# Autodesk Inventor assembly: PUERTA SP40-02 INT-EXT 2073x761
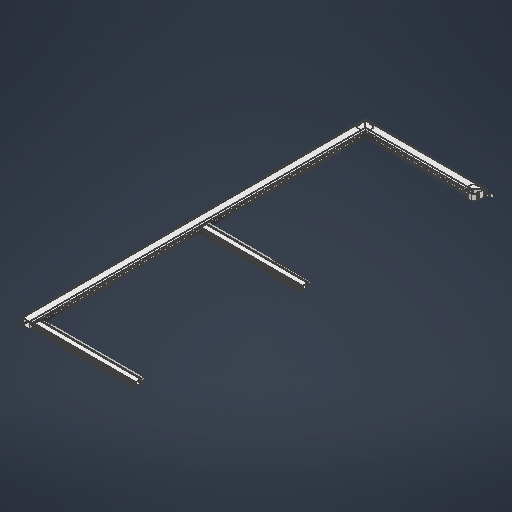
[picture p0: Inventor's stored thumbnail of the model, 512x512]
Saved by Autodesk Inventor 2025 (Build 290162000, 162)
## iProperties
Created: 2026-02-13
Part Number: PUERTA SP40-02 INT-EXT 2073x761
Document SubType Name: Assembly
Designer: ROLANDO
Author: ROLANDO
## Documents named in this file (16)
- C:\Users\rolan\OneDrive\Documentos\Inventor\Projects\CARPINTERIA ALUMINIO\PUERTAS Y VENTANAS\PUERTAS\PUERTA SP40-02 INT-EXT 2073x761.iam
- C:\Users\rolan\OneDrive\Documentos\Inventor\Projects\CARPINTERIA ALUMINIO\PUERTAS Y VENTANAS\PUERTAS\SP40-02 HOJA PUERTA BATIENTE INT - EXT 761 mm.ipt
- SP40-02 HOJA PUERTA BATIENTE INT - EXT 761 mm.ipt
- C:\Users\rolan\OneDrive\Documentos\Inventor\Projects\CARPINTERIA ALUMINIO\PUERTAS Y VENTANAS\PUERTAS\SP40-02 HOJA PUERTA BATIENTE INT - EXT 2073 mm.ipt
- SP40-02 HOJA PUERTA BATIENTE INT - EXT 2073 mm.ipt
- C:\Users\rolan\OneDrive\Documentos\Inventor\Projects\CARPINTERIA ALUMINIO\PUERTAS Y VENTANAS\ESCUADRAS\ESCUADRA UNIÓN 45 GRUESA.ipt
- C:\Users\rolan\OneDrive\Documentos\Inventor\Projects\CARPINTERIA ALUMINIO\PUERTAS Y VENTANAS\PUERTAS\SP40-02 JUNTA EXT 2073.ipt
- C:\Users\rolan\OneDrive\Documentos\Inventor\Projects\CARPINTERIA ALUMINIO\PUERTAS Y VENTANAS\PUERTAS\SP40-02 JUNTA EXT 761.ipt
- C:\Users\rolan\OneDrive\Documentos\Inventor\Projects\CARPINTERIA ALUMINIO\PUERTAS Y VENTANAS\PUERTAS\SP40-02 JUNTA INT 2073.ipt
- C:\Users\rolan\OneDrive\Documentos\Inventor\Projects\CARPINTERIA ALUMINIO\PUERTAS Y VENTANAS\PUERTAS\SP40-02 JUNTA INT 761.ipt
- C:\Users\rolan\OneDrive\Documentos\Inventor\Projects\CARPINTERIA ALUMINIO\PUERTAS Y VENTANAS\PUERTAS\SP40-02 HOJA PUERTA BATIENTE INT - EXT 2073 mm_MIR.ipt
- C:\Users\rolan\OneDrive\Documentos\Inventor\Projects\CARPINTERIA ALUMINIO\PUERTAS Y VENTANAS\PUERTAS\SP40-02 JUNTA EXT 2073_MIR.ipt
- C:\Users\rolan\OneDrive\Documentos\Inventor\Projects\CARPINTERIA ALUMINIO\PUERTAS Y VENTANAS\PUERTAS\SP40-02 JUNTA INT 2073_MIR.ipt
- C:\Users\rolan\OneDrive\Documentos\Inventor\Projects\CARPINTERIA ALUMINIO\PUERTAS Y VENTANAS\ESCUADRAS\ESCUADRA UNIÓN 45 GRUESA_MIR3.ipt
- C:\Users\rolan\OneDrive\Documentos\Inventor\Projects\CARPINTERIA ALUMINIO\PUERTAS Y VENTANAS\PUERTAS\SP40-04 TRAVESAÑO CENTRAL ZOCALO 602x60.ipt
- C:\Users\rolan\OneDrive\Documentos\Inventor\Projects\CARPINTERIA ALUMINIO\PUERTAS Y VENTANAS\PUERTAS\SP40-02 JUNTA INT 602 ZOCALO.ipt
## Components (16 placed, 13 different names)
1. SP40-02 HOJA PUERTA BATIENTE INT - EXT 761 mm:1 — Coincidencia:1, Coincidencia:3, Coincidencia:4, Coincidencia:5, Coincidencia:13, Coincidencia:14, Nivelación:5, Coincidencia:15, Coincidencia:16, Nivelación:6, Nivelación:9, Coincidencia:23, Coincidencia:25, Coincidencia:26, Coincidencia:29
2. SP40-02 HOJA PUERTA BATIENTE INT - EXT 2073 mm:1 — Coincidencia:2, Coincidencia:4, Coincidencia:5, Coincidencia:6, Coincidencia:7, Coincidencia:8, Nivelación:2, Coincidencia:11, Coincidencia:12, Nivelación:4
3. ESCUADRA UNIÓN 45 GRUESA:1 — Coincidencia:1, Coincidencia:2, Coincidencia:3, Coincidencia:6
4. SP40-02 JUNTA EXT 2073:1 — Coincidencia:7, Coincidencia:8, Nivelación:2
5. SP40-02 JUNTA EXT 761:1 — Coincidencia:15, Coincidencia:16, Nivelación:6
6. SP40-02 JUNTA INT 2073:1 — Coincidencia:11, Coincidencia:12, Nivelación:4
7. SP40-02 JUNTA INT 761:1 — Coincidencia:13, Coincidencia:14, Nivelación:5
8. SP40-02 HOJA PUERTA BATIENTE INT - EXT 2073 mm_MIR:1 — Coincidencia:18, Nivelación:7, Coincidencia:19, Coincidencia:20, Nivelación:8, Coincidencia:21, Coincidencia:22, Coincidencia:24, Coincidencia:25, Coincidencia:26, Coincidencia:27, Nivelación:10, Coincidencia:28, Nivelación:11, Nivelación:12
9. ESCUADRA UNIÓN 45 GRUESA_MIR3:1 — Nivelación:9, Coincidencia:18, Coincidencia:23, Coincidencia:24
10. SP40-02 JUNTA EXT 2073_MIR:1 — Nivelación:7, Coincidencia:19, Coincidencia:20
11. SP40-02 JUNTA INT 2073_MIR:1 — Nivelación:8, Coincidencia:21, Coincidencia:22
12. SP40-04 TRAVESAÑO CENTRAL ZOCALO 602x60:1 — Coincidencia:28, Nivelación:11, Nivelación:12, Coincidencia:30, Coincidencia:31, Nivelación:13
13. SP40-04 TRAVESAÑO CENTRAL ZOCALO 602x60:2 — Coincidencia:27, Nivelación:10, Coincidencia:29, Coincidencia:32, Coincidencia:33, Nivelación:14, Coincidencia:34, Coincidencia:35, Nivelación:15
14. SP40-02 JUNTA INT 602 ZOCALO:1 — Coincidencia:32, Coincidencia:33, Nivelación:14
15. SP40-02 JUNTA INT 602 ZOCALO:2 — Coincidencia:34, Coincidencia:35, Nivelación:15
16. SP40-02 JUNTA INT 602 ZOCALO:3 — Coincidencia:30, Coincidencia:31, Nivelación:13
## Relationships (45: Mate 32, Flush 13)
- Coincidencia:1 [Mate]: SP40-02 HOJA PUERTA BATIENTE INT - EXT 761 mm:1 ↔ ESCUADRA UNIÓN 45 GRUESA:1
- Coincidencia:2 [Mate]: SP40-02 HOJA PUERTA BATIENTE INT - EXT 2073 mm:1 ↔ ESCUADRA UNIÓN 45 GRUESA:1
- Coincidencia:3 [Mate] (0.2 mm): SP40-02 HOJA PUERTA BATIENTE INT - EXT 761 mm:1 ↔ ESCUADRA UNIÓN 45 GRUESA:1
- Coincidencia:4 [Mate]: SP40-02 HOJA PUERTA BATIENTE INT - EXT 761 mm:1 ↔ SP40-02 HOJA PUERTA BATIENTE INT - EXT 2073 mm:1
- Coincidencia:5 [Mate]: SP40-02 HOJA PUERTA BATIENTE INT - EXT 761 mm:1 ↔ SP40-02 HOJA PUERTA BATIENTE INT - EXT 2073 mm:1
- Coincidencia:6 [Mate] (0.1 mm): SP40-02 HOJA PUERTA BATIENTE INT - EXT 2073 mm:1 ↔ ESCUADRA UNIÓN 45 GRUESA:1
- Coincidencia:7 [Mate]: SP40-02 HOJA PUERTA BATIENTE INT - EXT 2073 mm:1 ↔ SP40-02 JUNTA EXT 2073:1
- Coincidencia:8 [Mate]: SP40-02 HOJA PUERTA BATIENTE INT - EXT 2073 mm:1 ↔ SP40-02 JUNTA EXT 2073:1
- Nivelación:2 [Flush]: SP40-02 HOJA PUERTA BATIENTE INT - EXT 2073 mm:1 ↔ SP40-02 JUNTA EXT 2073:1
- Coincidencia:11 [Mate]: SP40-02 HOJA PUERTA BATIENTE INT - EXT 2073 mm:1 ↔ SP40-02 JUNTA INT 2073:1
- Coincidencia:12 [Mate]: SP40-02 HOJA PUERTA BATIENTE INT - EXT 2073 mm:1 ↔ SP40-02 JUNTA INT 2073:1
- Nivelación:4 [Flush]: SP40-02 HOJA PUERTA BATIENTE INT - EXT 2073 mm:1 ↔ SP40-02 JUNTA INT 2073:1
- Coincidencia:13 [Mate]: SP40-02 HOJA PUERTA BATIENTE INT - EXT 761 mm:1 ↔ SP40-02 JUNTA INT 761:1
- Coincidencia:14 [Mate]: SP40-02 HOJA PUERTA BATIENTE INT - EXT 761 mm:1 ↔ SP40-02 JUNTA INT 761:1
- Nivelación:5 [Flush]: SP40-02 HOJA PUERTA BATIENTE INT - EXT 761 mm:1 ↔ SP40-02 JUNTA INT 761:1
- Coincidencia:15 [Mate]: SP40-02 HOJA PUERTA BATIENTE INT - EXT 761 mm:1 ↔ SP40-02 JUNTA EXT 761:1
- Coincidencia:16 [Mate]: SP40-02 HOJA PUERTA BATIENTE INT - EXT 761 mm:1 ↔ SP40-02 JUNTA EXT 761:1
- Nivelación:6 [Flush]: SP40-02 HOJA PUERTA BATIENTE INT - EXT 761 mm:1 ↔ SP40-02 JUNTA EXT 761:1
- Nivelación:9 [Flush]: SP40-02 HOJA PUERTA BATIENTE INT - EXT 761 mm:1 ↔ ESCUADRA UNIÓN 45 GRUESA_MIR3:1
- Coincidencia:18 [Mate]: SP40-02 HOJA PUERTA BATIENTE INT - EXT 2073 mm_MIR:1 ↔ ESCUADRA UNIÓN 45 GRUESA_MIR3:1
- Nivelación:7 [Flush]: SP40-02 HOJA PUERTA BATIENTE INT - EXT 2073 mm_MIR:1 ↔ SP40-02 JUNTA EXT 2073_MIR:1
- Coincidencia:19 [Mate]: SP40-02 HOJA PUERTA BATIENTE INT - EXT 2073 mm_MIR:1 ↔ SP40-02 JUNTA EXT 2073_MIR:1
- Coincidencia:20 [Mate]: SP40-02 HOJA PUERTA BATIENTE INT - EXT 2073 mm_MIR:1 ↔ SP40-02 JUNTA EXT 2073_MIR:1
- Nivelación:8 [Flush]: SP40-02 HOJA PUERTA BATIENTE INT - EXT 2073 mm_MIR:1 ↔ SP40-02 JUNTA INT 2073_MIR:1
- Coincidencia:21 [Mate]: SP40-02 HOJA PUERTA BATIENTE INT - EXT 2073 mm_MIR:1 ↔ SP40-02 JUNTA INT 2073_MIR:1
- Coincidencia:22 [Mate]: SP40-02 HOJA PUERTA BATIENTE INT - EXT 2073 mm_MIR:1 ↔ SP40-02 JUNTA INT 2073_MIR:1
- Coincidencia:23 [Mate] (0.2 mm): SP40-02 HOJA PUERTA BATIENTE INT - EXT 761 mm:1 ↔ ESCUADRA UNIÓN 45 GRUESA_MIR3:1
- Coincidencia:24 [Mate] (0.1 mm): SP40-02 HOJA PUERTA BATIENTE INT - EXT 2073 mm_MIR:1 ↔ ESCUADRA UNIÓN 45 GRUESA_MIR3:1
- Coincidencia:25 [Mate]: SP40-02 HOJA PUERTA BATIENTE INT - EXT 761 mm:1 ↔ SP40-02 HOJA PUERTA BATIENTE INT - EXT 2073 mm_MIR:1
- Coincidencia:26 [Mate]: SP40-02 HOJA PUERTA BATIENTE INT - EXT 761 mm:1 ↔ SP40-02 HOJA PUERTA BATIENTE INT - EXT 2073 mm_MIR:1
- Coincidencia:27 [Mate]: SP40-02 HOJA PUERTA BATIENTE INT - EXT 2073 mm_MIR:1 ↔ SP40-04 TRAVESAÑO CENTRAL ZOCALO 602x60:2
- Nivelación:10 [Flush]: SP40-02 HOJA PUERTA BATIENTE INT - EXT 2073 mm_MIR:1 ↔ SP40-04 TRAVESAÑO CENTRAL ZOCALO 602x60:2
- Coincidencia:28 [Mate]: SP40-02 HOJA PUERTA BATIENTE INT - EXT 2073 mm_MIR:1 ↔ SP40-04 TRAVESAÑO CENTRAL ZOCALO 602x60:1
- Nivelación:11 [Flush]: SP40-02 HOJA PUERTA BATIENTE INT - EXT 2073 mm_MIR:1 ↔ SP40-04 TRAVESAÑO CENTRAL ZOCALO 602x60:1
- Nivelación:12 [Flush]: SP40-02 HOJA PUERTA BATIENTE INT - EXT 2073 mm_MIR:1 ↔ SP40-04 TRAVESAÑO CENTRAL ZOCALO 602x60:1
- Coincidencia:29 [Mate] (930.25 mm): SP40-02 HOJA PUERTA BATIENTE INT - EXT 761 mm:1 ↔ SP40-04 TRAVESAÑO CENTRAL ZOCALO 602x60:2
- Coincidencia:30 [Mate]: SP40-04 TRAVESAÑO CENTRAL ZOCALO 602x60:1 ↔ SP40-02 JUNTA INT 602 ZOCALO:3
- Coincidencia:31 [Mate]: SP40-04 TRAVESAÑO CENTRAL ZOCALO 602x60:1 ↔ SP40-02 JUNTA INT 602 ZOCALO:3
- Nivelación:13 [Flush]: SP40-04 TRAVESAÑO CENTRAL ZOCALO 602x60:1 ↔ SP40-02 JUNTA INT 602 ZOCALO:3
- Coincidencia:32 [Mate]: SP40-04 TRAVESAÑO CENTRAL ZOCALO 602x60:2 ↔ SP40-02 JUNTA INT 602 ZOCALO:1
- Coincidencia:33 [Mate]: SP40-04 TRAVESAÑO CENTRAL ZOCALO 602x60:2 ↔ SP40-02 JUNTA INT 602 ZOCALO:1
- Nivelación:14 [Flush]: SP40-04 TRAVESAÑO CENTRAL ZOCALO 602x60:2 ↔ SP40-02 JUNTA INT 602 ZOCALO:1
- Coincidencia:34 [Mate]: SP40-04 TRAVESAÑO CENTRAL ZOCALO 602x60:2 ↔ SP40-02 JUNTA INT 602 ZOCALO:2
- Coincidencia:35 [Mate]: SP40-04 TRAVESAÑO CENTRAL ZOCALO 602x60:2 ↔ SP40-02 JUNTA INT 602 ZOCALO:2
- Nivelación:15 [Flush]: SP40-04 TRAVESAÑO CENTRAL ZOCALO 602x60:2 ↔ SP40-02 JUNTA INT 602 ZOCALO:2
